# Autodesk Inventor assembly: SSE2B-MX10-455
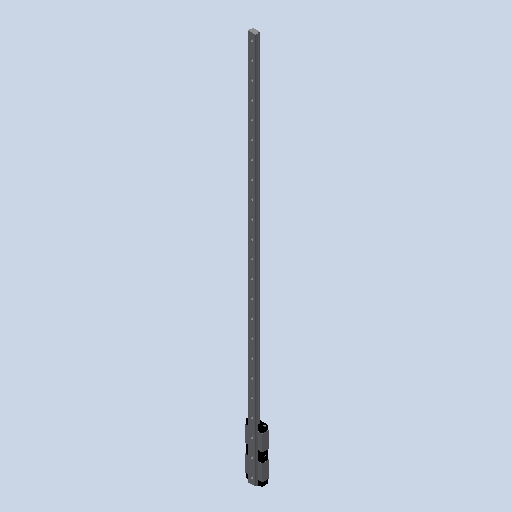
[picture p0: Inventor's stored thumbnail of the model, 512x512]
Saved by Autodesk Inventor 2025.1 (Build 291241000, 241)
## iProperties
Category: PARTsolutions
Company: MISUMI
Created: 2024-08-09
Part Number: SSE2B-MX10-455
Catalog Web Link: www.cadenas.de
Description: SSEB, SSEB-MX, SSE2B, SSE2B-MX, RSEB, RSE2B-Miniature Linear Guides Standard Blocks/Light Preload High Grade-L Selectable Type
Vendor: MISUMI
Document SubType Name: Assembly
Designer: psAdmin
Manufacturer: MISUMI
Mass: 25.2481 g
Surface Area: 211.952 cm^2
Volume: 25.2481 cm^3
PSOL_IDENT_0: {$CADENAS_DATA/23d-libs/misumi/metric/06_linear_guides/re2b_asmtab.prj},265 {VTYP=3D},{STYP=ASSTAB},
PSOL_IDENT_1: {NB=SSE2B-MX10-455},{LINA=SSE2B-MX10-455},{NN=SSEB, SSEB-MX, SSE2B, SSE2B-MX, RSEB, RSE2B},{DATE=04.
PSOL_IDENT_2: 04.2024 07:12:35},{GEOMDATE=07.03.2024 00:33:43},{VERSION=},{LINEID=160},{WBVAR=ST,MAT,MX,NOB,GREASE
PSOL_IDENT_3: ,LS,ALT1,ALT2,ALT3,ALT4},{WBNUMERIC=LS}  {NB=SSE2B-MX10-455},{LINA=SSE2B-MX10-455},{KT=DUMMY},{PN=SS
PSOL_IDENT_4: E2B-MX10-455},{RT=B},{TYPE=SSE2B},{ST=S},{MAT=S},{MX=-MX},{MXALG='', 'w/o MX(Lubrication unit)', '-M
PSOL_IDENT_5: X', 'with MX(Lubrication unit)'},{NOB=2},{H=10},{GREASE=},{GREASEALG='','Normal'},{LT=Selectable},{L
PSOL_IDENT_6: S=455},{HARD=56HRC~},{W=20},{L1=30.0},{B=15},{C=10},{SLL=M3x3},{L2=19.0},{K=7.8},{CBB=0.3},{W1=9},{W
PSOL_IDENT_7: 2=5.5},{H1=5.5},{CAA=0.3},{DD1DD2HH=3.5x6x3.5},{F=20},{G=7.5},{ALT1=},{ALT1ALG= '', 'w/o MC (Tapped
PSOL_IDENT_8: Holes)' },{MC=M4},{ALT2=},{ALT2L=2.5},{ALT2N=5},{M=23},{LL=},{L0=75,95,115,135,155,175,195,215,235,2
PSOL_IDENT_9: 55,275,295,315,335,355,355,375,395,415,435,455,475,495,515,535,555,575,595,615,635},{REC1=   '','w/o
PSOL_IDENT_10: Rail Ends Cut alteration','-LLC','with LLC (Left End Cut)','-RLC','with RLC (Right End Cut)','-LLC-
PSOL_IDENT_11: RLC','with Both End Cut'   },{ST1='S', 'w/o Surface Treatment'},{MAT2='S','Stainless Steel'},{ALT3=}
PSOL_IDENT_12: ,{ALT3ALG= '' , 'w/o WC (Pair of Rails)'},{ALT4=},{ALT4ALG= '','N/A' },{PPATH=seb_series/seb_asmtpl.
PSOL_IDENT_13: prj}
NB: SSE2B-MX10-455
NN: SSEB, SSEB-MX, SSE2B, SSE2B-MX, RSEB, RSE2B
NT: Miniature Linear Guides Standard Blocks/Light Preload High Grade-L Selectable Type
NBSYN: $PN.
LINA: SSE2B-MX10-455
CATALOG: Misumi
PN: SSE2B-MX10-455
ST: w/o Surface Treatment
MAT: Stainless Steel
MX: with MX(Lubrication unit)
NOB: 2
H: 10
GREASE: Normal
LS: 455
W: 20
L1: 30
B: 15
C: 10
SLL: M3x3
L2: 19
K: 7.8
CBB: 0.3
W1: 9
W2: 5.5
H1: 5.5
CAA: 0.3
DD1DD2HH: 3.5x6x3.5
F: 20
G: 7.5
ALT1: w/o MC (Tapped Holes)
ALT2: w/o Rail Ends Cut alteration
ALT3: w/o WC (Pair of Rails)
ALT4: N/A
SUPPLIER: MISUMI
ARTICLENO: SSE2B-MX10-455
BOMINFO: SSE2B-MX10-455
CREATOR: CADENAS GmbH
Title: SSE2B-MX10-455
Author: Cadenas PARTsolutions
Comments: Miniature Linear Guides Standard Blocks/Light Preload High Grade-L Selectable Type
## Documents named in this file (3)
- C:\Users\haruy\Documents\ロボコン\NHK2025\cad\nagahisa\belt_liner\SSE2B-MX10-455.iam
- C:\Users\haruy\Documents\ロボコン\NHK2025\cad\nagahisa\belt_liner\SSE2B-MX10-455_r.ipt
- C:\Users\haruy\Documents\ロボコン\NHK2025\cad\nagahisa\belt_liner\SSEB-MX10_b.ipt
## Components (3 placed, 2 different names)
1. SSE2B-MX10-455_r:1 — to_block_Z@1 <-> to_rail_Z@2, to_block_YZ@1 <-> to_rail_YZ@2, to_block_2_Z@1 <-> to_rail_Z@3, to_block_2_YZ@1 <-> to_rail_YZ@3
2. SSEB-MX10_b:1 — to_block_Z@1 <-> to_rail_Z@2, to_block_YZ@1 <-> to_rail_YZ@2, メイト:3
3. SSEB-MX10_b:2 — to_block_2_Z@1 <-> to_rail_Z@3, to_block_2_YZ@1 <-> to_rail_YZ@3, メイト:3
## Relationships (5: Mate 3, Angle 2)
- to_block_Z@1 <-> to_rail_Z@2 [Mate]: SSE2B-MX10-455_r:1 ↔ SSEB-MX10_b:1
- to_block_YZ@1 <-> to_rail_YZ@2 [Angle] (0 deg): SSE2B-MX10-455_r:1 ↔ SSEB-MX10_b:1
- to_block_2_Z@1 <-> to_rail_Z@3 [Mate]: SSE2B-MX10-455_r:1 ↔ SSEB-MX10_b:2
- to_block_2_YZ@1 <-> to_rail_YZ@3 [Angle] (0 deg): SSE2B-MX10-455_r:1 ↔ SSEB-MX10_b:2
- メイト:3 [Mate]: SSEB-MX10_b:1 ↔ SSEB-MX10_b:2
